# Autodesk Inventor assembly: Belt Tensioner 10mm
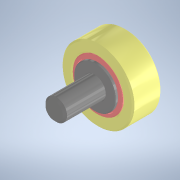
[picture p0: Inventor's stored thumbnail of the model, 180x180]
Saved by Autodesk Inventor 2022.2 (Build 262287000, 287)
## iProperties
Created: 2022-01-06
Part Number: Belt Tensioner 10mm
Document SubType Name: Assembly
Designer: Jochen
Author: Jochen
## Documents named in this file (5)
- D:\Projects\Chewbacca\CAD\Common\Belt Tensioner\Belt Tensioner 10mm.iam
- D:\Projects\Chewbacca\CAD\Common\Belt Tensioner\TransmissionBeltTensionerRoller.ipt
- D:\Projects\Chewbacca\inspiration\open_robot_actuator_hardware-master\mechanics\quadruped_robot_12dof_v1\solidworks_files\quadruped_12dof_v1\fastener_washer_m2.5.ipt
- D:\Projects\Chewbacca\CAD\Common\Bearing\bearing_7_3_3_sbn_683_2ZVA.ipt
- D:\Projects\Chewbacca\CAD\Common\Fastener\fastener_fhs_m3_10.ipt
## Components (4 placed, 4 different names)
1. Belt Tensioner 10mm:1 — Mate:1, Mate:4, Mate:6, Mate:7
2. fastener_washer_m2.5:1 — Mate:3, Mate:5
3. bearing_7_3_3_sbn_683_2ZVA:1 — Mate:1, Mate:2, Mate:5, Mate:6, Mate:7
4. fastener_fhs_m3_10:1 — Mate:2, Mate:3, Mate:4
## Relationships (7: Mate 7)
- Mate:1: Belt Tensioner 10mm:1 ↔ bearing_7_3_3_sbn_683_2ZVA:1
- Mate:2: bearing_7_3_3_sbn_683_2ZVA:1 ↔ fastener_fhs_m3_10:1
- Mate:3: fastener_washer_m2.5:1 ↔ fastener_fhs_m3_10:1
- Mate:4: Belt Tensioner 10mm:1 ↔ fastener_fhs_m3_10:1
- Mate:5: fastener_washer_m2.5:1 ↔ bearing_7_3_3_sbn_683_2ZVA:1
- Mate:6: Belt Tensioner 10mm:1 ↔ bearing_7_3_3_sbn_683_2ZVA:1
- Mate:7: Belt Tensioner 10mm:1 ↔ bearing_7_3_3_sbn_683_2ZVA:1
